# Autodesk Inventor assembly: PutTogether
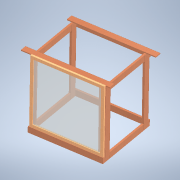
[picture p0: Inventor's stored thumbnail of the model, 180x180]
Saved by Autodesk Inventor 2020 (Build 240168000, 168)
## iProperties
Created: 2020-05-19
Part Number: PutTogether
Document SubType Name: Assembly
Designer: kolbe
Author: kolbe
## Documents named in this file (3)
- C:\Users\kolbe\Documents\GitHub\Terrarium\PutTogether.iam
- C:\Users\kolbe\Documents\GitHub\Terrarium\structure\wood structure.iam
- C:\Users\kolbe\Documents\GitHub\Terrarium\door\door_w_glass.iam
## Components (2 placed, 2 different names)
1. wood structure:1 [sub-assembly] — Planar:1
2. door_w_glass:1 [sub-assembly] — Planar:1
## Relationships (1: PlanarJoint 1)
- Planar:1: wood structure:1 ↔ door_w_glass:1
